# Autodesk Inventor assembly: AddOn_Module
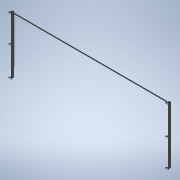
[picture p0: Inventor's stored thumbnail of the model, 180x180]
Saved by Autodesk Inventor 2021 (Build 250183000, 183)
## iProperties
Created: 2021-04-05
Part Number: AddOn_Module
Document SubType Name: Assembly
Designer: Jorian Brusind
Author: Jorian Brusind
## Documents named in this file (8)
- C:\Users\Jorian Bruslind\Documents\GitHub\PersonalProjects\HyperRail\Inventor Files\AddOn_Module.iam
- C:\Users\Jorian Bruslind\Documents\GitHub\PersonalProjects\Inventor Projects\Useful models\8020_Sets\IPT_40_Series\Extra_40_Series\HFS5-4060-4000\HFS5-4060-2125.ipt
- C:\Users\Jorian Bruslind\Documents\GitHub\PersonalProjects\HyperRail\Inventor Files\SDP_sdpsi_a_6r25mc250\SDP_sdpsi_a_6r25mc1000.ipt
- C:\Users\Jorian Bruslind\Documents\GitHub\PersonalProjects\HyperRail\Inventor Files\Bottom_Foot_Standoff.ipt
- C:\Users\Jorian Bruslind\Documents\GitHub\PersonalProjects\HyperRail\Inventor Files\SpacerBlock_25mm.ipt
- C:\Users\Jorian Bruslind\Documents\GitHub\PersonalProjects\HyperRail\Inventor Files\McMaster Files\Leveling Feet\62805K49_Heavy Duty Leveling Mount.ipt
- C:\Users\Jorian Bruslind\Documents\GitHub\PersonalProjects\HyperRail\Inventor Files\SpacingStrut.iam
- C:\Users\Jorian Bruslind\Documents\GitHub\PersonalProjects\HyperRail\Inventor Files\Metric bolt\Bolt M5 40mm.ipt
## Components (37 placed, 7 different names)
1. HFS5-4060-2125:1 — Mate:35, Flush:40, Mate:59, Mate:60, Flush:43, Mate:62
2. SDP_sdpsi_a_6r25mc1000:1
3. SDP_sdpsi_a_6r25mc1000:2
4. Bottom_Foot_Standoff:1 — Mate:66, Mate:68
5. SpacerBlock_25mm:1
6. 62805K49_Heavy Duty Leveling Mount:1
7. 62805K49_Heavy Duty Leveling Mount:2
8. Bottom_Foot_Standoff:2 — Mate:65, Mate:67
9. SpacerBlock_25mm:2
10. 62805K49_Heavy Duty Leveling Mount:3 — Mate:34
11. 62805K49_Heavy Duty Leveling Mount:4
12. Bottom_Foot_Standoff:3 — Mate:63, Mate:64
13. SpacerBlock_25mm:3
14. 62805K49_Heavy Duty Leveling Mount:5
15. 62805K49_Heavy Duty Leveling Mount:6
16. HFS5-4060-2125:2 — Flush:40, Mate:60, Flush:41, Mate:61
17. SDP_sdpsi_a_6r25mc1000:3
18. SDP_sdpsi_a_6r25mc1000:4
19. Bottom_Foot_Standoff:4 — Mate:69, Mate:74
20. SpacerBlock_25mm:4
21. 62805K49_Heavy Duty Leveling Mount:7
22. 62805K49_Heavy Duty Leveling Mount:8
23. Bottom_Foot_Standoff:5 — Mate:70, Mate:73
24. SpacerBlock_25mm:5
25. 62805K49_Heavy Duty Leveling Mount:9
26. 62805K49_Heavy Duty Leveling Mount:10
27. Bottom_Foot_Standoff:6 — Mate:71, Mate:72
28. SpacerBlock_25mm:6
29. 62805K49_Heavy Duty Leveling Mount:11
30. 62805K49_Heavy Duty Leveling Mount:12
31. SpacingStrut:1 [sub-assembly] — Mate:59, Flush:41, Mate:61, Flush:43, Mate:62
32. Bolt M5 40mm:1 — Mate:63, Mate:64
33. Bolt M5 40mm:2 — Mate:65, Mate:67
34. Bolt M5 40mm:3 — Mate:66, Mate:68
35. Bolt M5 40mm:4 — Mate:71, Mate:72
36. Bolt M5 40mm:5 — Mate:70, Mate:73
37. Bolt M5 40mm:6 — Mate:69, Mate:74
## Relationships (95: Mate 60, Flush 35)
- [Flush]: SDP_sdpsi_a_6r25mc1000:1 ↔ SDP_sdpsi_a_6r25mc1000:2
- [Mate]: SDP_sdpsi_a_6r25mc1000:1 ↔ SDP_sdpsi_a_6r25mc1000:2
- [Flush]: SDP_sdpsi_a_6r25mc1000:1 ↔ SDP_sdpsi_a_6r25mc1000:2
- [Mate] (1 mm): HFS5-4060-2125:1 ↔ SDP_sdpsi_a_6r25mc1000:1
- [Flush]: HFS5-4060-2125:1 ↔ SDP_sdpsi_a_6r25mc1000:1
- [Flush]: HFS5-4060-2125:1 ↔ SDP_sdpsi_a_6r25mc1000:1
- [Flush]: HFS5-4060-2125:1 ↔ Bottom_Foot_Standoff:1
- [Mate]: HFS5-4060-2125:1 ↔ SpacerBlock_25mm:1
- [Flush]: HFS5-4060-2125:1 ↔ SpacerBlock_25mm:1
- [Flush] (20 mm): HFS5-4060-2125:1 ↔ SpacerBlock_25mm:1
- [Mate]: Bottom_Foot_Standoff:1 ↔ SpacerBlock_25mm:1
- [Mate]: Bottom_Foot_Standoff:1 ↔ SpacerBlock_25mm:1
- [Flush]: Bottom_Foot_Standoff:1 ↔ SpacerBlock_25mm:1
- [Mate]: Bottom_Foot_Standoff:1 ↔ 62805K49_Heavy Duty Leveling Mount:1
- [Mate]: Bottom_Foot_Standoff:1 ↔ 62805K49_Heavy Duty Leveling Mount:2
- [Flush]: 62805K49_Heavy Duty Leveling Mount:1 ↔ 62805K49_Heavy Duty Leveling Mount:2
- [Mate] (20 mm): Bottom_Foot_Standoff:1 ↔ 62805K49_Heavy Duty Leveling Mount:1
- [Mate]: Bottom_Foot_Standoff:2 ↔ SpacerBlock_25mm:2
- [Mate]: Bottom_Foot_Standoff:2 ↔ SpacerBlock_25mm:2
- [Flush]: Bottom_Foot_Standoff:2 ↔ SpacerBlock_25mm:2
- [Mate]: Bottom_Foot_Standoff:2 ↔ 62805K49_Heavy Duty Leveling Mount:3
- [Mate]: Bottom_Foot_Standoff:2 ↔ 62805K49_Heavy Duty Leveling Mount:4
- [Flush]: 62805K49_Heavy Duty Leveling Mount:3 ↔ 62805K49_Heavy Duty Leveling Mount:4
- [Mate] (20 mm): Bottom_Foot_Standoff:2 ↔ 62805K49_Heavy Duty Leveling Mount:3
- [Mate]: Bottom_Foot_Standoff:3 ↔ SpacerBlock_25mm:3
- [Mate]: Bottom_Foot_Standoff:3 ↔ SpacerBlock_25mm:3
- [Flush]: Bottom_Foot_Standoff:3 ↔ SpacerBlock_25mm:3
- [Mate]: Bottom_Foot_Standoff:3 ↔ 62805K49_Heavy Duty Leveling Mount:5
- [Mate]: Bottom_Foot_Standoff:3 ↔ 62805K49_Heavy Duty Leveling Mount:6
- [Flush]: 62805K49_Heavy Duty Leveling Mount:5 ↔ 62805K49_Heavy Duty Leveling Mount:6
- [Mate] (20 mm): Bottom_Foot_Standoff:3 ↔ 62805K49_Heavy Duty Leveling Mount:5
- [Mate]: HFS5-4060-2125:1 ↔ SpacerBlock_25mm:3
- [Mate]: HFS5-4060-2125:1 ↔ SpacerBlock_25mm:2
- [Flush]: HFS5-4060-2125:1 ↔ SpacerBlock_25mm:3
- [Flush] (20 mm): HFS5-4060-2125:1 ↔ SpacerBlock_25mm:3
- [Flush] (20 mm): HFS5-4060-2125:1 ↔ SpacerBlock_25mm:2
- [Mate] (1000 mm): SpacerBlock_25mm:2 ↔ SpacerBlock_25mm:3
- Mate:34: 62805K49_Heavy Duty Leveling Mount:3
- Mate:35: HFS5-4060-2125:1
- [Flush]: SDP_sdpsi_a_6r25mc1000:3 ↔ SDP_sdpsi_a_6r25mc1000:4
- [Mate]: SDP_sdpsi_a_6r25mc1000:3 ↔ SDP_sdpsi_a_6r25mc1000:4
- [Flush]: SDP_sdpsi_a_6r25mc1000:3 ↔ SDP_sdpsi_a_6r25mc1000:4
- [Mate] (1 mm): HFS5-4060-2125:2 ↔ SDP_sdpsi_a_6r25mc1000:3
- [Flush]: HFS5-4060-2125:2 ↔ SDP_sdpsi_a_6r25mc1000:3
- [Flush]: HFS5-4060-2125:2 ↔ SDP_sdpsi_a_6r25mc1000:3
- [Flush]: HFS5-4060-2125:2 ↔ Bottom_Foot_Standoff:4
- [Mate]: HFS5-4060-2125:2 ↔ SpacerBlock_25mm:4
- [Flush]: HFS5-4060-2125:2 ↔ SpacerBlock_25mm:4
- [Flush] (20 mm): HFS5-4060-2125:2 ↔ SpacerBlock_25mm:4
- [Mate]: Bottom_Foot_Standoff:4 ↔ SpacerBlock_25mm:4
- [Mate]: Bottom_Foot_Standoff:4 ↔ SpacerBlock_25mm:4
- [Flush]: Bottom_Foot_Standoff:4 ↔ SpacerBlock_25mm:4
- [Mate]: Bottom_Foot_Standoff:4 ↔ 62805K49_Heavy Duty Leveling Mount:7
- [Mate]: Bottom_Foot_Standoff:4 ↔ 62805K49_Heavy Duty Leveling Mount:8
- [Flush]: 62805K49_Heavy Duty Leveling Mount:7 ↔ 62805K49_Heavy Duty Leveling Mount:8
- [Mate] (20 mm): Bottom_Foot_Standoff:4 ↔ 62805K49_Heavy Duty Leveling Mount:7
- [Mate]: Bottom_Foot_Standoff:5 ↔ SpacerBlock_25mm:5
- [Mate]: Bottom_Foot_Standoff:5 ↔ SpacerBlock_25mm:5
- [Flush]: Bottom_Foot_Standoff:5 ↔ SpacerBlock_25mm:5
- [Mate]: Bottom_Foot_Standoff:5 ↔ 62805K49_Heavy Duty Leveling Mount:9
- [Mate]: Bottom_Foot_Standoff:5 ↔ 62805K49_Heavy Duty Leveling Mount:10
- [Flush]: 62805K49_Heavy Duty Leveling Mount:9 ↔ 62805K49_Heavy Duty Leveling Mount:10
- [Mate] (20 mm): Bottom_Foot_Standoff:5 ↔ 62805K49_Heavy Duty Leveling Mount:9
- [Mate]: Bottom_Foot_Standoff:6 ↔ SpacerBlock_25mm:6
- [Mate]: Bottom_Foot_Standoff:6 ↔ SpacerBlock_25mm:6
- [Flush]: Bottom_Foot_Standoff:6 ↔ SpacerBlock_25mm:6
- [Mate]: Bottom_Foot_Standoff:6 ↔ 62805K49_Heavy Duty Leveling Mount:11
- [Mate]: Bottom_Foot_Standoff:6 ↔ 62805K49_Heavy Duty Leveling Mount:12
- [Flush]: 62805K49_Heavy Duty Leveling Mount:11 ↔ 62805K49_Heavy Duty Leveling Mount:12
- [Mate] (20 mm): Bottom_Foot_Standoff:6 ↔ 62805K49_Heavy Duty Leveling Mount:11
- [Mate]: HFS5-4060-2125:2 ↔ SpacerBlock_25mm:6
- [Mate]: HFS5-4060-2125:2 ↔ SpacerBlock_25mm:5
- [Flush]: HFS5-4060-2125:2 ↔ SpacerBlock_25mm:6
- [Flush] (20 mm): HFS5-4060-2125:2 ↔ SpacerBlock_25mm:6
- [Flush] (20 mm): HFS5-4060-2125:2 ↔ SpacerBlock_25mm:5
- [Mate] (1000 mm): SpacerBlock_25mm:5 ↔ SpacerBlock_25mm:6
- Flush:40: HFS5-4060-2125:1 ↔ HFS5-4060-2125:2
- Mate:59 (-20 mm): HFS5-4060-2125:1 ↔ SpacingStrut:1
- Mate:60 (5793 mm): HFS5-4060-2125:1 ↔ HFS5-4060-2125:2
- Flush:41: HFS5-4060-2125:2 ↔ SpacingStrut:1
- Mate:61: HFS5-4060-2125:2 ↔ SpacingStrut:1
- Flush:43: HFS5-4060-2125:1 ↔ SpacingStrut:1
- Mate:62: HFS5-4060-2125:1 ↔ SpacingStrut:1
- Mate:63: Bottom_Foot_Standoff:3 ↔ Bolt M5 40mm:1
- Mate:64: Bottom_Foot_Standoff:3 ↔ Bolt M5 40mm:1
- Mate:65: Bottom_Foot_Standoff:2 ↔ Bolt M5 40mm:2
- Mate:66: Bottom_Foot_Standoff:1 ↔ Bolt M5 40mm:3
- Mate:67: Bottom_Foot_Standoff:2 ↔ Bolt M5 40mm:2
- Mate:68: Bottom_Foot_Standoff:1 ↔ Bolt M5 40mm:3
- Mate:69: Bottom_Foot_Standoff:4 ↔ Bolt M5 40mm:6
- Mate:70: Bottom_Foot_Standoff:5 ↔ Bolt M5 40mm:5
- Mate:71: Bottom_Foot_Standoff:6 ↔ Bolt M5 40mm:4
- Mate:72: Bottom_Foot_Standoff:6 ↔ Bolt M5 40mm:4
- Mate:73: Bottom_Foot_Standoff:5 ↔ Bolt M5 40mm:5
- Mate:74: Bottom_Foot_Standoff:4 ↔ Bolt M5 40mm:6
## Named parameters: d763_d759 = 0 mm, d764_d760 = 0 mm, d765_d761 = 0 mm, d766_d762 = 20 mm, d767_d752 = 0 mm, d768_d753 = 0 mm, d769_d754 = 0 mm, d770_d759 = 0 mm, d771_d760 = 0 mm, d772_d761 = 0 mm, d773_d762 = 20 mm, d774_d752 = 0 mm, d775_d753 = 0 mm, d776_d754 = 0 mm, d66_d746 = 0 mm, d67_d749 = 0 mm, d68_d750 = 0 mm, d69_d751 = 20 mm, d70_d752 = 0 mm, d71_d753 = 0 mm, d72_d754 = 0 mm, d73_d759 = 0 mm, d74_d760 = 0 mm, d75_d761 = 0 mm, d76_d762 = 20 mm, d77_d763_d759 = 0 mm, d78_d764_d760 = 0 mm, d79_d765_d761 = 0 mm, d80_d766_d762 = 20 mm, d81_d767_d752 = 0 mm, d82_d768_d753 = 0 mm, d83_d769_d754 = 0 mm, d84_d770_d759 = 0 mm, d85_d771_d760 = 0 mm, d86_d772_d761 = 0 mm, d87_d773_d762 = 20 mm, d88_d774_d752 = 0 mm, d89_d775_d753 = 0 mm, d90_d776_d754 = 0 mm, d91_d777 = 0 mm, d92_d778 = 0 mm, d93_d779 = 0 mm, d94_d780 = 20 mm, d95_d781 = 20 mm, d96_d782 = 1000 mm, d97_d633 = 0 mm, d98_d634 = 0 mm, d99_d635 = 0 mm, d100_d636 = 1 mm, d101_d637 = 0 mm, d102_d638 = 0 mm
